# Autodesk Inventor assembly: assembled
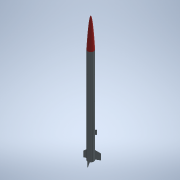
[picture p0: Inventor's stored thumbnail of the model, 180x180]
Saved by Autodesk Inventor 2020.3 (Build 243373000, 373)
## iProperties
Created: 2021-03-15
Part Number: assembled
Document SubType Name: Assembly
Designer: 0x6f736f646f
Author: 0x6f736f646f
## Documents named in this file (8)
- C:\Users\0x6f736f646f\OneDrive\Documents\Nakuja\airframev1\Design\assembled.iam
- C:\Users\0x6f736f646f\OneDrive\Documents\Nakuja\airframev1\Design\noseAssembly.iam
- C:\Users\0x6f736f646f\OneDrive\Documents\Nakuja\airframev1\Design\electronicsbay.ipt
- C:\Users\0x6f736f646f\OneDrive\Documents\Nakuja\airframev1\Design\extraTube.ipt
- C:\Users\0x6f736f646f\OneDrive\Documents\Nakuja\airframev1\Design\launchlug.ipt
- C:\Users\0x6f736f646f\OneDrive\Documents\Nakuja\airframev1\Design\payloadchamber.ipt
- C:\Users\0x6f736f646f\OneDrive\Documents\Nakuja\airframev1\Design\tail.ipt
- C:\Users\0x6f736f646f\OneDrive\Documents\Nakuja\airframev1\Design\motor-mount-bottom.ipt
## Components (8 placed, 7 different names)
1. extraTube:1 — Mate:1, Mate:2
2. launchlug:1 — Mate:6, Mate:7
3. noseAssembly:1 [sub-assembly] — Insert:2
4. payloadchamber:1 — Insert:1, Insert:2, Mate:1
5. tail:1 — Mate:3, Mate:4, Mate:5, Mate:6, Mate:7
6. extraTube:2 — Mate:2, Mate:3
7. motor-mount-bottom:1 — Mate:4, Mate:5
8. electronicsbay:1 — Insert:1
## Relationships (9: Mate 7, Insert 2)
- Insert:1: payloadchamber:1 ↔ electronicsbay:1
- Insert:2: noseAssembly:1 ↔ payloadchamber:1
- Mate:1: extraTube:1 ↔ payloadchamber:1
- Mate:2: extraTube:1 ↔ extraTube:2
- Mate:3: tail:1 ↔ extraTube:2
- Mate:4: tail:1 ↔ motor-mount-bottom:1
- Mate:5: tail:1 ↔ motor-mount-bottom:1
- Mate:6 (33.6 mm): launchlug:1 ↔ tail:1
- Mate:7: launchlug:1 ↔ tail:1
